# Autodesk Inventor assembly: Leg
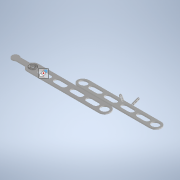
[picture p0: Inventor's stored thumbnail of the model, 180x180]
Saved by Autodesk Inventor 2022 (Build 260153000, 153)
## iProperties
Created: 2022-03-17
Part Number: Leg
Document SubType Name: Assembly
Designer: br4ch
Author: br4ch
## Documents named in this file (5)
- C:\Users\br4ch\M-and-Ms\Strirus\Leg.iam
- C:\Users\br4ch\M-and-Ms\Strirus\psmall.ipt
- C:\Users\br4ch\M-and-Ms\Strirus\p2.ipt
- C:\Users\br4ch\M-and-Ms\Strirus\p1.ipt
- C:\Users\br4ch\M-and-Ms\Strirus\Leg\Design Accelerator\Bearing2.iam
## Components (5 placed, 4 different names)
1. psmall:1
2. psmall:2
3. p2:1
4. p1:1 — Mate:1, Mate:2
5. Bearing:1 [sub-assembly] — Mate:1, Mate:2
## Relationships (2: Mate 2)
- Mate:1: p1:1 ↔ Bearing:1
- Mate:2: p1:1 ↔ Bearing:1
